# Autodesk Inventor assembly: Gimbal Assembly
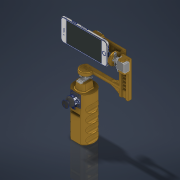
[picture p0: Inventor's stored thumbnail of the model, 180x180]
Saved by Autodesk Inventor 2022 (Build 260153000, 153)
## iProperties
Created: 2021-07-30
Part Number: Gimbal Assembly
Document SubType Name: Assembly
Designer: sidsa
Author: sidsa
## Documents named in this file (7)
- D:\My Documents\gitHUB Rocketry\mlh-selfie-hacks\CAD Models\Gimbal Assembly.iam
- D:\My Documents\gitHUB Rocketry\mlh-selfie-hacks\CAD Models\Mg90 Servo\MG90servo_assembly.ipt
- D:\My Documents\gitHUB Rocketry\mlh-selfie-hacks\CAD Models\iPhone\iphone 6.ipt
- D:\My Documents\gitHUB Rocketry\mlh-selfie-hacks\CAD Models\Roll Pitch Axis Support.ipt
- D:\My Documents\gitHUB Rocketry\mlh-selfie-hacks\CAD Models\Yaw Axis Support.ipt
- D:\My Documents\gitHUB Rocketry\mlh-selfie-hacks\CAD Models\Joystick\Joystick HW504 Board.ipt
- D:\My Documents\gitHUB Rocketry\mlh-selfie-hacks\CAD Models\Handle.ipt
## Components (8 placed, 6 different names)
1. MG90servo_assembly:3 — Flush:2, Flush:3, Mate:9, Mate:13, Mate:14, Mate:15, Mate:16
2. iphone 6:1 — Mate:1
3. MG90servo_assembly:4 — Mate:1, Mate:2, Flush:1, Mate:3, Flush:2
4. MG90servo_assembly:5 — Mate:4, Mate:5, Mate:6, Mate:7, Mate:8, Flush:3
5. Roll Pitch Axis Support:1 — Mate:2, Flush:1, Mate:3, Mate:4, Mate:5
6. Yaw Axis Support:1 — Mate:6, Mate:7, Mate:8, Mate:9
7. Joystick HW504 Board:1 — Mate:10, Mate:11, Mate:12
8. Handle:1 — Mate:10, Mate:11, Mate:12, Mate:13, Mate:14, Mate:15, Mate:16
## Relationships (19: Mate 16, Flush 3)
- Mate:1: iphone 6:1 ↔ MG90servo_assembly:4
- Mate:2: MG90servo_assembly:4 ↔ Roll Pitch Axis Support:1
- Flush:1: MG90servo_assembly:4 ↔ Roll Pitch Axis Support:1
- Mate:3: MG90servo_assembly:4 ↔ Roll Pitch Axis Support:1
- Mate:4: MG90servo_assembly:5 ↔ Roll Pitch Axis Support:1
- Mate:5: MG90servo_assembly:5 ↔ Roll Pitch Axis Support:1
- Mate:6: MG90servo_assembly:5 ↔ Yaw Axis Support:1
- Flush:2: MG90servo_assembly:3 ↔ MG90servo_assembly:4
- Mate:7: MG90servo_assembly:5 ↔ Yaw Axis Support:1
- Mate:8: MG90servo_assembly:5 ↔ Yaw Axis Support:1
- Flush:3: MG90servo_assembly:3 ↔ MG90servo_assembly:5
- Mate:9: MG90servo_assembly:3 ↔ Yaw Axis Support:1
- Mate:10: Joystick HW504 Board:1 ↔ Handle:1
- Mate:11: Joystick HW504 Board:1 ↔ Handle:1
- Mate:12: Joystick HW504 Board:1 ↔ Handle:1
- Mate:13: MG90servo_assembly:3 ↔ Handle:1
- Mate:14: MG90servo_assembly:3 ↔ Handle:1
- Mate:15: MG90servo_assembly:3 ↔ Handle:1
- Mate:16: MG90servo_assembly:3 ↔ Handle:1
